# Autodesk Inventor assembly: AssemblyVero
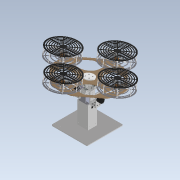
[picture p0: Inventor's stored thumbnail of the model, 180x180]
Saved by Autodesk Inventor 2021.1 (Build 251245010, 245A)
## iProperties
Created: 2023-10-22
Part Number: AssemblyVero
Document SubType Name: Assembly
Designer: M
Author: M
## Documents named in this file (4)
- F:\College\Semester_9\GP\Cad\hover231125\Workspaces\Workspace\AssemblyVero.iam
- F:\College\Semester_9\GP\Cad\hover231125\Workspaces\Workspace\Base_V2.iam
- F:\College\Semester_9\GP\Cad\hover231125\Workspaces\Workspace\SecondJoint.iam
- F:\College\Semester_9\GP\Cad\hover231125\Workspaces\Workspace\FirstJoint.iam
## Components (3 placed, 3 different names)
1. Base_V2:1 [sub-assembly] — Mate:1, Mate:3, Flush:3, Mate:4, Mate:5
2. SecondJoint:1 [sub-assembly] — Mate:2, Flush:2, Angle:2, Angle:3
3. FirstJoint:1 [sub-assembly] — Mate:1, Mate:2, Flush:2, Mate:3, Angle:1, Angle:3
## Relationships (10: Mate 5, Angle 3, Flush 2)
- Mate:1: Base_V2:1 ↔ FirstJoint:1
- Mate:2: SecondJoint:1 ↔ FirstJoint:1
- Flush:2 (-30 mm): SecondJoint:1 ↔ FirstJoint:1
- Mate:3 (3 mm): Base_V2:1 ↔ FirstJoint:1
- Angle:1 (180 deg): FirstJoint:1
- Angle:2 (180 deg): SecondJoint:1
- Flush:3: Base_V2:1
- Mate:4: Base_V2:1
- Mate:5: Base_V2:1
- Angle:3 (0 deg): SecondJoint:1 ↔ FirstJoint:1
